# Autodesk Inventor assembly: YAxisMotorLeft
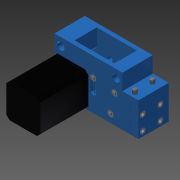
[picture p0: Inventor's stored thumbnail of the model, 180x180]
Saved by Autodesk Inventor 2015 (Build 190159000, 159)
## iProperties
Created: 2014-08-09
Part Number: YAxisMotorLeft
Document SubType Name: Assembly
Designer: Jack
Author: Jack
## Documents named in this file (13)
- C:\Users\Jack\ownCloud\Projects\CoreXY\InventorModel\Old\YAxis\YAxisMotor\YAxisMotorLeft.old.iam
- C:\Users\Jack\ownCloud\Projects\CoreXY\InventorModel\Old\YAxis\YAxisMotor\YAxisMotorBlock.old.ipt
- C:\Users\Jack\ownCloud\Projects\CoreXY\InventorModel\Old\YAxis\YAxisMotor\YAxisMotorCap.old.ipt
- C:\Users\Jack\ownCloud\Projects\CoreXY\InventorModel\Hardware\Bolts\SHCS\SHCS5\SHCS5x10.ipt
- C:\Users\Jack\ownCloud\Projects\CoreXY\InventorModel\Hardware\Bolts\FHS\FHS5\5x10FHS.ipt
- C:\Users\Jack\ownCloud\Projects\CoreXY\InventorModel\Hardware\Bolts\SHCS\SHCS4\SHCS4x35.ipt
- C:\Users\Jack\ownCloud\Projects\CoreXY\InventorModel\Hardware\Bolts\SHCS\SHCS3\SHCS3x8.ipt
- C:\Users\Jack\ownCloud\Projects\CoreXY\InventorModel\Electronics\Motors\StepperMotorNema17.ipt
- C:\Users\Jack\ownCloud\Projects\CoreXY\InventorModel\Hardware\Bolts\SHCS\SHCS4\SHCS4x15.ipt
- C:\Users\Jack\ownCloud\Projects\CoreXY\InventorModel\Hardware\Nuts\Nut4.ipt
- C:\Users\Jack\ownCloud\Projects\CoreXY\InventorModel\Hardware\Belt\PulleyGT2x20tx5mmBore.ipt
- C:\Users\Jack\ownCloud\Projects\CoreXY\InventorModel\Hardware\Bearing\BearingRadialBall\BearingRadialBallF624zz.ipt
- C:\Users\Jack\ownCloud\Projects\CoreXY\InventorModel\Hardware\Wahsers\M4Washer.ipt
## Components (39 placed, 12 different names)
1. YAxisMotorBlock.old:1 — Mate:1, Flush:1, Mate:2, Mate:3, Mate:4, Mate:5, Mate:6, Flush:2, Mate:7, Mate:8, Mate:9, Mate:10, Mate:11, Flush:3, Mate:12, Mate:13, Mate:14, Mate:15, Mate:16, Slider:1, Mate:17, Mate:18, Mate:19, Mate:20, Mate:21, Mate:22, Mate:23, Mate:24, Mate:25, Flush:4, Mate:39, Mate:40, Mate:41, Angle:1, Angle:2, Angle:3, Flush:5, Mate:58, Mate:66, Mate:74, Mate:75, Mate:76, Mate:77, Mate:78, Angle:4, Angle:5, Angle:6, Angle:7
2. YAxisMotorCap.old:1 — Mate:1, Flush:1, Flush:4, Mate:28, Mate:29, Mate:30, Mate:31, Mate:32, Mate:33, Mate:34, Mate:35
3. StepperMotorNema17:1 — Mate:25, Mate:26, Mate:27, Mate:50
4. PulleyGT2x20tx5mmBore:1 — Mate:50, Flush:5
5. SHCS4x35:1 — Mate:13, Mate:16, Mate:36, Mate:57
6. Nut4:3 — Mate:36, Mate:41, Angle:1
7. Nut4:4 — Mate:37, Mate:40, Angle:2
8. SHCS4x35:2 — Mate:14, Mate:15, Mate:37, Mate:65
9. Nut4:5 — Mate:38, Mate:39, Angle:3
10. SHCS4x35:3 — Slider:1, Mate:38, Mate:73
11. M4Washer:1
12. M4Washer:2 — Mate:57, Mate:58
13. M4Washer:5
14. M4Washer:6 — Mate:73, Mate:74
15. M4Washer:3
16. M4Washer:4 — Mate:65, Mate:66
17. BearingRadialBallF624zz:1
18. BearingRadialBallF624zz:2
19. BearingRadialBallF624zz:3
20. BearingRadialBallF624zz:4
21. BearingRadialBallF624zz:5
22. BearingRadialBallF624zz:6
23. SHCS4x15:1 — Mate:30, Mate:34, Mate:44
24. SHCS4x15:2 — Mate:31, Mate:35, Mate:43
25. SHCS4x15:3 — Mate:29, Mate:33, Mate:48
26. SHCS4x15:4 — Mate:28, Mate:32, Mate:46
27. Nut4:1 — Mate:48, Mate:78, Angle:4
28. Nut4:2 — Mate:46, Mate:77, Angle:5
29. Nut4:6 — Mate:44, Mate:75, Angle:7
30. Nut4:7 — Mate:43, Mate:76, Angle:6
31. SHCS5x10:2 — Mate:3, Mate:5
32. SHCS5x10:1 — Mate:2, Mate:4
33. 5x10FHS:1 — Mate:6, Flush:2
34. SHCS5x10:3 — Mate:7, Mate:9
35. SHCS5x10:4 — Mate:8, Mate:10
36. SHCS3x8:1 — Mate:17, Mate:24, Mate:26
37. SHCS3x8:2 — Mate:19, Mate:22
38. SHCS3x8:3 — Mate:18, Mate:23, Mate:27
39. SHCS3x8:4 — Mate:20, Mate:21
## Relationships (87: Mate 74, Angle 7, Flush 5, TranslationJoint 1)
- Mate:1: YAxisMotorBlock.old:1 ↔ YAxisMotorCap.old:1
- Flush:1: YAxisMotorBlock.old:1 ↔ YAxisMotorCap.old:1
- Mate:2: YAxisMotorBlock.old:1 ↔ SHCS5x10:1
- Mate:3: YAxisMotorBlock.old:1 ↔ SHCS5x10:2
- Mate:4: YAxisMotorBlock.old:1 ↔ SHCS5x10:1
- Mate:5: YAxisMotorBlock.old:1 ↔ SHCS5x10:2
- Mate:6: YAxisMotorBlock.old:1 ↔ 5x10FHS:1
- Flush:2: YAxisMotorBlock.old:1 ↔ 5x10FHS:1
- Mate:7: YAxisMotorBlock.old:1 ↔ SHCS5x10:3
- Mate:8: YAxisMotorBlock.old:1 ↔ SHCS5x10:4
- Mate:9: YAxisMotorBlock.old:1 ↔ SHCS5x10:3
- Mate:10: YAxisMotorBlock.old:1 ↔ SHCS5x10:4
- Mate:11: YAxisMotorBlock.old:1
- Flush:3: YAxisMotorBlock.old:1
- Mate:12: YAxisMotorBlock.old:1
- Mate:13: YAxisMotorBlock.old:1 ↔ SHCS4x35:1
- Mate:14: YAxisMotorBlock.old:1 ↔ SHCS4x35:2
- Mate:15: YAxisMotorBlock.old:1 ↔ SHCS4x35:2
- Mate:16: YAxisMotorBlock.old:1 ↔ SHCS4x35:1
- Slider:1 [TranslationJoint]: YAxisMotorBlock.old:1 ↔ SHCS4x35:3
- Mate:17: YAxisMotorBlock.old:1 ↔ SHCS3x8:1
- Mate:18: YAxisMotorBlock.old:1 ↔ SHCS3x8:3
- Mate:19: YAxisMotorBlock.old:1 ↔ SHCS3x8:2
- Mate:20: YAxisMotorBlock.old:1 ↔ SHCS3x8:4
- Mate:21: YAxisMotorBlock.old:1 ↔ SHCS3x8:4
- Mate:22: YAxisMotorBlock.old:1 ↔ SHCS3x8:2
- Mate:23: YAxisMotorBlock.old:1 ↔ SHCS3x8:3
- Mate:24: YAxisMotorBlock.old:1 ↔ SHCS3x8:1
- Mate:25: YAxisMotorBlock.old:1 ↔ StepperMotorNema17:1
- Mate:26: StepperMotorNema17:1 ↔ SHCS3x8:1
- Mate:27: StepperMotorNema17:1 ↔ SHCS3x8:3
- Flush:4: YAxisMotorBlock.old:1 ↔ YAxisMotorCap.old:1
- Mate:28: YAxisMotorCap.old:1 ↔ SHCS4x15:4
- Mate:29: YAxisMotorCap.old:1 ↔ SHCS4x15:3
- Mate:30: YAxisMotorCap.old:1 ↔ SHCS4x15:1
- Mate:31: YAxisMotorCap.old:1 ↔ SHCS4x15:2
- Mate:32: YAxisMotorCap.old:1 ↔ SHCS4x15:4
- Mate:33: YAxisMotorCap.old:1 ↔ SHCS4x15:3
- Mate:34: YAxisMotorCap.old:1 ↔ SHCS4x15:1
- Mate:35: YAxisMotorCap.old:1 ↔ SHCS4x15:2
- Mate:36: SHCS4x35:1 ↔ Nut4:3
- Mate:37: Nut4:4 ↔ SHCS4x35:2
- Mate:38: Nut4:5 ↔ SHCS4x35:3
- Mate:39: YAxisMotorBlock.old:1 ↔ Nut4:5
- Mate:40: YAxisMotorBlock.old:1 ↔ Nut4:4
- Mate:41: YAxisMotorBlock.old:1 ↔ Nut4:3
- Angle:1 (0 deg): YAxisMotorBlock.old:1 ↔ Nut4:3
- Angle:2 (0 deg): YAxisMotorBlock.old:1 ↔ Nut4:4
- Angle:3 (0 deg): YAxisMotorBlock.old:1 ↔ Nut4:5
- Mate:43: SHCS4x15:2 ↔ Nut4:7
- Mate:44: SHCS4x15:1 ↔ Nut4:6
- Mate:46: SHCS4x15:4 ↔ Nut4:2
- Mate:48: SHCS4x15:3 ↔ Nut4:1
- Mate:50: StepperMotorNema17:1 ↔ PulleyGT2x20tx5mmBore:1
- Flush:5 (-2.3 mm): YAxisMotorBlock.old:1 ↔ PulleyGT2x20tx5mmBore:1
- [Mate]: BearingRadialBallF624zz:1 ↔ BearingRadialBallF624zz:2
- [Mate]: BearingRadialBallF624zz:1 ↔ BearingRadialBallF624zz:2
- [Mate]: M4Washer:1 ↔ BearingRadialBallF624zz:1
- [Mate]: M4Washer:1 ↔ BearingRadialBallF624zz:2
- [Mate]: M4Washer:2 ↔ BearingRadialBallF624zz:1
- [Mate]: M4Washer:2 ↔ BearingRadialBallF624zz:1
- Mate:57: SHCS4x35:1 ↔ M4Washer:2
- Mate:58: YAxisMotorBlock.old:1 ↔ M4Washer:2
- [Mate]: BearingRadialBallF624zz:3 ↔ BearingRadialBallF624zz:4
- [Mate]: BearingRadialBallF624zz:3 ↔ BearingRadialBallF624zz:4
- [Mate]: M4Washer:3 ↔ BearingRadialBallF624zz:3
- [Mate]: M4Washer:3 ↔ BearingRadialBallF624zz:4
- [Mate]: M4Washer:4 ↔ BearingRadialBallF624zz:3
- [Mate]: M4Washer:4 ↔ BearingRadialBallF624zz:3
- Mate:65: SHCS4x35:2 ↔ M4Washer:4
- Mate:66: YAxisMotorBlock.old:1 ↔ M4Washer:4
- [Mate]: BearingRadialBallF624zz:5 ↔ BearingRadialBallF624zz:6
- [Mate]: BearingRadialBallF624zz:5 ↔ BearingRadialBallF624zz:6
- [Mate]: M4Washer:5 ↔ BearingRadialBallF624zz:5
- [Mate]: M4Washer:5 ↔ BearingRadialBallF624zz:6
- [Mate]: M4Washer:6 ↔ BearingRadialBallF624zz:5
- [Mate]: M4Washer:6 ↔ BearingRadialBallF624zz:5
- Mate:73: SHCS4x35:3 ↔ M4Washer:6
- Mate:74: YAxisMotorBlock.old:1 ↔ M4Washer:6
- Mate:75: YAxisMotorBlock.old:1 ↔ Nut4:6
- Mate:76: YAxisMotorBlock.old:1 ↔ Nut4:7
- Mate:77: YAxisMotorBlock.old:1 ↔ Nut4:2
- Mate:78: YAxisMotorBlock.old:1 ↔ Nut4:1
- Angle:4 (0 deg): YAxisMotorBlock.old:1 ↔ Nut4:1
- Angle:5 (0 deg): YAxisMotorBlock.old:1 ↔ Nut4:2
- Angle:6 (0 deg): YAxisMotorBlock.old:1 ↔ Nut4:7
- Angle:7 (0 deg): YAxisMotorBlock.old:1 ↔ Nut4:6
## Named parameters: d116_d160 = 0 mm, d117_d161 = 0 mm, d118_d162 = 0 mm, d119_d163 = 0 mm, d120_d158 = 0 mm, d121_d159 = 0 mm, d124_d160 = 0 mm, d125_d161 = 0 mm, d126_d162 = 0 mm, d127_d163 = 0 mm, d128_d158 = 0 mm, d129_d159 = 0 mm
